# Autodesk Inventor assembly: assemblage_nema8_gauche
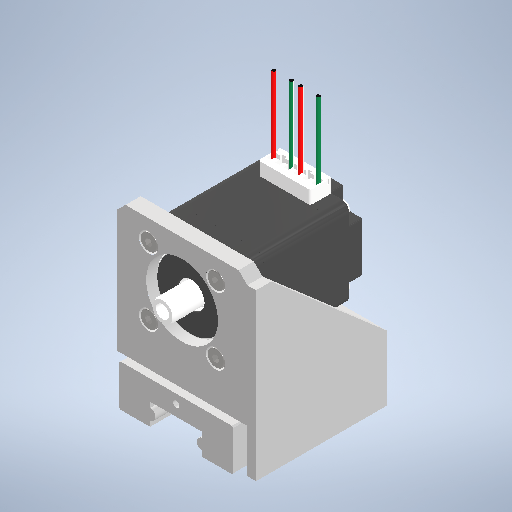
[picture p0: Inventor's stored thumbnail of the model, 512x512]
Saved by Autodesk Inventor 2025.1 (Build 291241000, 241)
## iProperties
Created: 2025-03-24
Part Number: assemblage_nema8_gauche
Document SubType Name: Assembly
Designer: felix
Author: felix
## Documents named in this file (6)
- D:\documents\projets inventor\Skibbidi Startech\assemblage_nema8_gauche.iam
- D:\documents\projets inventor\Skibbidi Startech\mgn12c_02.ipt
- C:\Users\felix\OneDrive - Haute Ecole de Namur-Liege-Luxembourg\Documents\Inventor\Content Center Files\R2025\fr-FR\BS EN ISO 4762\BS EN ISO 4762 - M3 x 10(1).ipt
- D:\documents\projets inventor\Skibbidi Startech\moteur_nema8.ipt
- C:\Users\felix\OneDrive - Haute Ecole de Namur-Liege-Luxembourg\Documents\Inventor\Content Center Files\R2025\fr-FR\BS EN ISO 4762\BS EN ISO 4762 - M2 x 5(1).ipt
- D:\documents\projets inventor\Skibbidi Startech\support nema8_gauche.ipt
## Components (11 placed, 5 different names)
1. mgn12c_02:1
2. BS EN ISO 4762 : Pièce 1 Vis cylindrique à six pans creux - Métrique M3 x 10:1
3. BS EN ISO 4762 : Pièce 1 Vis cylindrique à six pans creux - Métrique M3 x 10:2
4. BS EN ISO 4762 : Pièce 1 Vis cylindrique à six pans creux - Métrique M3 x 10:3
5. BS EN ISO 4762 : Pièce 1 Vis cylindrique à six pans creux - Métrique M3 x 10:4
6. moteur_nema8:1 — Placage:1, Placage:2
7. BS EN ISO 4762 : Pièce 1 Vis cylindrique à six pans creux - Métrique M2 x 5:1
8. BS EN ISO 4762 : Pièce 1 Vis cylindrique à six pans creux - Métrique M2 x 5:2
9. BS EN ISO 4762 : Pièce 1 Vis cylindrique à six pans creux - Métrique M2 x 5:3
10. BS EN ISO 4762 : Pièce 1 Vis cylindrique à six pans creux - Métrique M2 x 5:4
11. support nema8_gauche:1 — Placage:1, Placage:2
## Relationships (2: Mate 2)
- Placage:1 [Mate]: moteur_nema8:1 ↔ support nema8_gauche:1
- Placage:2 [Mate]: moteur_nema8:1 ↔ support nema8_gauche:1
